# Autodesk Inventor assembly: assemble_ver5
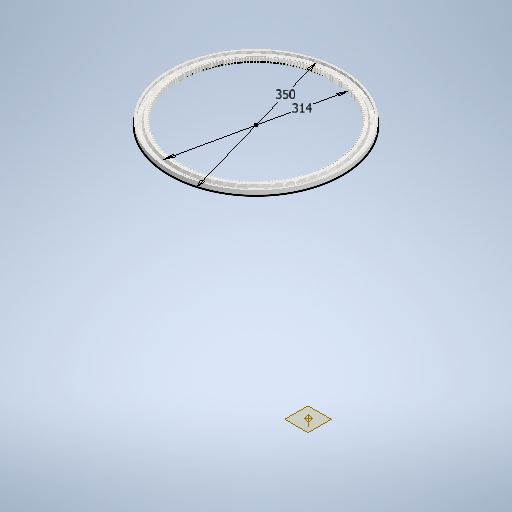
[picture p0: Inventor's stored thumbnail of the model, 512x512]
Saved by Autodesk Inventor 2025 (Build 290162000, 162)
## iProperties
Created: 2025-12-09
Part Number: assemble_ver5
Document SubType Name: Assembly
Designer: Admin
Author: Admin
## Documents named in this file (4)
- C:\Users\sum89\OneDrive\Рабочий стол\Ring\Model\assemble_ver5.iam
- C:\Users\sum89\OneDrive\Рабочий стол\Ring\Model\assemble_ver5\Мастер проектирования\Цилиндрическое зубчатое зацепление1.iam
- C:\Users\sum89\OneDrive\Рабочий стол\Ring\Model\assemble_ver4.ipt
- C:\Users\sum89\OneDrive\Рабочий стол\Ring\Model\assemble_ver5\Мастер проектирования\Цилиндрическое зубчатое зацепление2.iam
## Components (3 placed, 2 different names)
1. Цилиндрическое зубчатое зацепление:1 [sub-assembly] — Совмещение:1, Совмещение:2, Совмещение:3, Угол:1
2. assemble_ver4:1 — Совмещение:6, Заподлицо:1
3. Цилиндрическое зубчатое зацепление:2 [sub-assembly] — Совмещение:6, Заподлицо:1
## Relationships (8: Mate 6, Angle 1, Flush 1)
- Совмещение:1 [Mate]: Цилиндрическое зубчатое зацепление:1
- Совмещение:2 [Mate]: Цилиндрическое зубчатое зацепление:1
- Совмещение:3 [Mate]: Цилиндрическое зубчатое зацепление:1
- Совмещение:4 [Mate]
- Совмещение:5 [Mate]
- Угол:1 [Angle] (0 deg): Цилиндрическое зубчатое зацепление:1
- Совмещение:6 [Mate]: assemble_ver4:1 ↔ Цилиндрическое зубчатое зацепление:2
- Заподлицо:1 [Flush]: assemble_ver4:1 ↔ Цилиндрическое зубчатое зацепление:2
